# Autodesk Inventor assembly: левый привод_MIR1
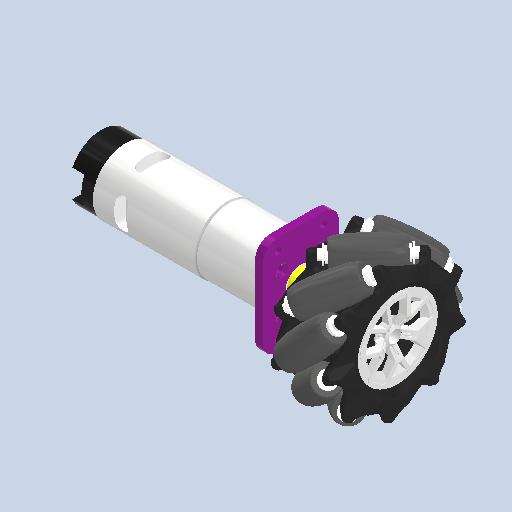
[picture p0: Inventor's stored thumbnail of the model, 512x512]
Saved by Autodesk Inventor 2025 (Build 290162000, 162)
## iProperties
Created: 2025-02-16
Part Number: левый привод_MIR1
Document SubType Name: Assembly
Designer: volko
Author: volko
## Documents named in this file (5)
- C:\Users\volko\Desktop\диплом\Модели\детали\левый привод_MIR1.iam
- C:\Users\volko\Desktop\диплом\Модели\детали\CHP-42GP-775 ABHL_MIR_MIR1.ipt
- C:\Users\volko\Desktop\диплом\Модели\детали\кронштейн_MIR_MIR1.ipt
- C:\Users\volko\Desktop\диплом\Модели\детали\переходная втулка_MIR_MIR1.ipt
- C:\Users\volko\Desktop\диплом\Модели\Mecanum wheel - left\Mecanum wheel - left_MIR1.iam
## Components (4 placed, 4 different names)
1. CHP-42GP-775 ABHL_MIR_MIR1:1 — Заподлицо:1, Совмещение:2, Совмещение:1, Совмещение:11, Совмещение:7, Совмещение:5, Совмещение:4, Совмещение:3
2. кронштейн_MIR_MIR1:1 — Совмещение:11, Совмещение:7, Совмещение:5
3. переходная втулка_MIR_MIR1:1 — Совмещение:4, Совмещение:3, Совмещение:10, Совмещение:9, Совмещение:8
4. Mecanum wheel - left_MIR1:1 [sub-assembly] — Совмещение:12, Совмещение:10, Совмещение:9, Совмещение:8
## Relationships (12: Mate 10, Flush 2)
- Заподлицо:1 [Flush]: CHP-42GP-775 ABHL_MIR_MIR1:1
- Совмещение:2 [Mate]: CHP-42GP-775 ABHL_MIR_MIR1:1
- Совмещение:1 [Mate]: CHP-42GP-775 ABHL_MIR_MIR1:1
- Совмещение:11 [Mate]: CHP-42GP-775 ABHL_MIR_MIR1:1 ↔ кронштейн_MIR_MIR1:1
- Совмещение:7 [Mate]: CHP-42GP-775 ABHL_MIR_MIR1:1 ↔ кронштейн_MIR_MIR1:1
- Совмещение:5 [Mate]: CHP-42GP-775 ABHL_MIR_MIR1:1 ↔ кронштейн_MIR_MIR1:1
- Совмещение:4 [Mate]: CHP-42GP-775 ABHL_MIR_MIR1:1 ↔ переходная втулка_MIR_MIR1:1
- Совмещение:3 [Mate]: CHP-42GP-775 ABHL_MIR_MIR1:1 ↔ переходная втулка_MIR_MIR1:1
- Совмещение:12 [Flush]: Mecanum wheel - left_MIR1:1
- Совмещение:10 [Mate]: переходная втулка_MIR_MIR1:1 ↔ Mecanum wheel - left_MIR1:1
- Совмещение:9 [Mate]: переходная втулка_MIR_MIR1:1 ↔ Mecanum wheel - left_MIR1:1
- Совмещение:8 [Mate]: переходная втулка_MIR_MIR1:1 ↔ Mecanum wheel - left_MIR1:1
